# Autodesk Inventor assembly: Plate pulley v 2.0
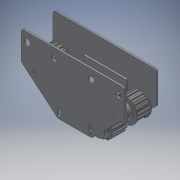
[picture p0: Inventor's stored thumbnail of the model, 180x180]
Saved by Autodesk Inventor 2016 (Build 200138000, 138)
## iProperties
Created: 2015-10-10
Part Number: Plate pulley v 2.0
Document SubType Name: Assembly
Designer: Delta
Author: Delta
## Documents named in this file (7)
- C:\Robotics\2015-16_CAD\custom cad parts\Plate pulley v 2.0.iam
- C:\Robotics\2015-16_CAD\custom cad parts\Hex standoff custom.ipt
- C:\Robotics\2015-16_CAD\custom cad parts\track side panel V1 - screw hole edition.ipt
- C:\Robotics\2015-16_CAD\custom cad parts\track side panel V1 - top hole edidtion .ipt
- C:\Robotics\2015-16_CAD\custom cad parts\wheel and axel top.iam
- C:\Robotics\2015-16_CAD\custom cad parts\wheel and axel bottom.iam
- E:\Autodesk CAD\track bracket.ipt
## Components (8 placed, 6 different names)
1. Hex standoff custom:2 — Insert:5
2. track side panel V1 - screw hole edition:1 — Flush:1, Insert:7
3. track side panel V1 - top hole edidtion :1 — Insert:1, Insert:2, Insert:3, Insert:4, Insert:5, Flush:1, Insert:6, Mate:1
4. wheel and axel top:1 [sub-assembly] — Insert:1
5. wheel and axel top:2 [sub-assembly] — Insert:2
6. wheel and axel bottom:1 [sub-assembly] — Insert:3
7. wheel and axel bottom:2 [sub-assembly] — Insert:4
8. track bracket:1 — Insert:6, Mate:1, Insert:7
## Relationships (9: Insert 7, Flush 1, Mate 1)
- Insert:1: track side panel V1 - top hole edidtion :1 ↔ wheel and axel top:1
- Insert:2: track side panel V1 - top hole edidtion :1 ↔ wheel and axel top:2
- Insert:3: track side panel V1 - top hole edidtion :1 ↔ wheel and axel bottom:1
- Insert:4: track side panel V1 - top hole edidtion :1 ↔ wheel and axel bottom:2
- Insert:5: Hex standoff custom:2 ↔ track side panel V1 - top hole edidtion :1
- Flush:1: track side panel V1 - screw hole edition:1 ↔ track side panel V1 - top hole edidtion :1
- Insert:6: track side panel V1 - top hole edidtion :1 ↔ track bracket:1
- Mate:1: track side panel V1 - top hole edidtion :1 ↔ track bracket:1
- Insert:7: track side panel V1 - screw hole edition:1 ↔ track bracket:1
